# Autodesk Inventor assembly: brace
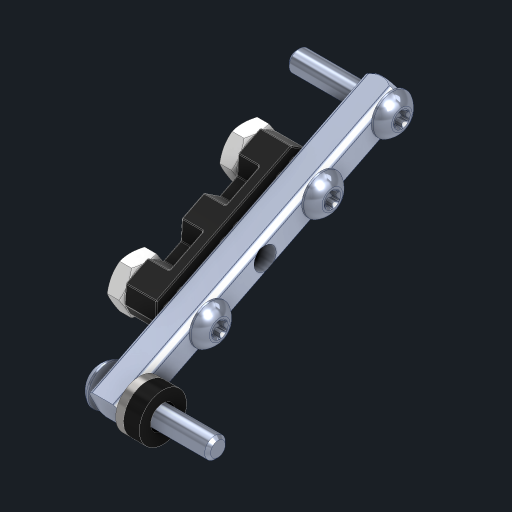
[picture p0: Inventor's stored thumbnail of the model, 512x512]
Saved by Autodesk Inventor 2024 (Build 280153000, 153)
## iProperties
Created: 2023-08-22
Part Number: brace
Document SubType Name: Assembly
Designer: Averey
Author: Averey
## Documents named in this file (13)
- C:\Users\Averey\Documents\vex\cad\scrap_v0.1\catapult\brace.iam
- C:\Users\Averey\Documents\vex\cad\scrap_v0.1\catapult\custom_parts\hs_brace.ipt
- C:\Users\Averey\Documents\vex\cad\VEX-CAD-Inventor-1.41\Motion\Shaft LS\Bearing Flat Low Profile.ipt
- C:\Users\Averey\Documents\vex\cad\VEX-CAD-Inventor-1.41\Structure\Hardware\Screw Steel - Star\SScrew Star Smooth .625.ipt
- C:\Users\Averey\Documents\vex\cad\VEX-CAD-Inventor-1.41\Structure\Hardware\Screw Steel - Star.ipt
- C:\Users\Averey\Documents\vex\cad\VEX-CAD-Inventor-1.41\Structure\Hardware\Nut Nylon\Nut Nylon - White.ipt
- C:\Users\Averey\Documents\vex\cad\VEX-CAD-Inventor-1.41\Structure\Hardware\Nut Nylon.ipt
- C:\Users\Averey\Documents\vex\cad\VEX-CAD-Inventor-1.41\Motion\Spacers\Spacer Nylon .375 OD\NSpacer .375 OD x .125.ipt
- C:\Users\Averey\Documents\vex\cad\VEX-CAD-Inventor-1.41\Motion\Spacers\Spacer Nylon .375 OD.ipt
- C:\Users\Averey\Documents\vex\cad\VEX-CAD-Inventor-1.41\Motion\Spacers\Washer Steel\SWasher .375 OD x .062500.ipt
- C:\Users\Averey\Documents\vex\cad\VEX-CAD-Inventor-1.41\Motion\Spacers\Washer Steel.ipt
- C:\Users\Averey\Documents\vex\cad\VEX-CAD-Inventor-1.41\Structure\Hardware\Screw Steel - Star\SScrew Star Smooth .750.ipt
- C:\Users\Averey\Documents\vex\cad\VEX-CAD-Inventor-1.41\Structure\Hardware\Screw Steel - Star\SScrew Star Smooth .875.ipt
## Components (10 placed, 8 different names)
1. hs_brace:1 — Insert:2, Insert:3, Insert:7, Insert:8, Insert:9
2. Bearing Flat Low Profile:1 — Insert:4, Insert:5
3. SScrew Star Smooth .625:1 — Insert:3
4. SScrew Star Smooth .625:2 — Insert:2
5. Nut Nylon - White:1 — Insert:5
6. Nut Nylon - White:2 — Insert:4
7. NSpacer .375 OD x .125:1 — Insert:6
8. SWasher .375 OD x .062500:1 — Insert:6, Insert:7
9. SScrew Star Smooth .750:3 — Insert:8
10. SScrew Star Smooth .875:4 — Insert:9
## Relationships (10: Insert 9, Mate 1)
- [Insert]: hs_brace:1 ↔ Bearing Flat Low Profile:1
- [Mate]: hs_brace:1 ↔ Bearing Flat Low Profile:1
- Insert:2: hs_brace:1 ↔ SScrew Star Smooth .625:2
- Insert:3: hs_brace:1 ↔ SScrew Star Smooth .625:1
- Insert:4 (1.27 mm): Bearing Flat Low Profile:1 ↔ Nut Nylon - White:2
- Insert:5 (1.27 mm): Bearing Flat Low Profile:1 ↔ Nut Nylon - White:1
- Insert:6: NSpacer .375 OD x .125:1 ↔ SWasher .375 OD x .062500:1
- Insert:7: hs_brace:1 ↔ SWasher .375 OD x .062500:1
- Insert:8: hs_brace:1 ↔ SScrew Star Smooth .750:3
- Insert:9: hs_brace:1 ↔ SScrew Star Smooth .875:4
